# Autodesk Inventor assembly: power_pcb.brd
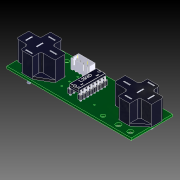
[picture p0: Inventor's stored thumbnail of the model, 180x180]
Saved by Autodesk Inventor 2020 (Build 240168000, 168)
## iProperties
Created: 2021-08-06
Part Number: power_pcb.brd
Document SubType Name: Assembly
Designer: Петров Иван
Mass: 15.8912 g
Surface Area: 154.202 cm^2
Volume: 15.8912 cm^3
Density: 1 g/cm^3
Author: Петров Иван
## Documents named in this file (6)
- E:\IVAN\Ivan_desktop\Kvantorium\Projects\RoboPatrol\electronic\COMMUATOR_POWER_PCB\power_pcb.brd.iam
- E:\IVAN\Ivan_desktop\Kvantorium\Projects\RoboPatrol\design\standart_components\BR05-PCB.ipt
- E:\IVAN\Ivan_desktop\Kvantorium\Projects\RoboPatrol\design\standart_components\SCSL-4.ipt
- E:\IVAN\Ivan_desktop\Kvantorium\Projects\RoboPatrol\design\standart_components\L293D v1.ipt
- E:\IVAN\Ivan_desktop\Kvantorium\Projects\RoboPatrol\design\standart_components\connectrs\JST - XH - Thru (V) - 4Pin - 2.54mm.ipt
- E:\IVAN\Ivan_desktop\Kvantorium\Projects\RoboPatrol\electronic\COMMUATOR_POWER_PCB\power_pcb.brdКонтур1.ipt
## Components (9 placed, 5 different names)
1. power_pcb.brdКонтур:2
2. BR05-PCB:1
3. BR05-PCB:2
4. L293D v1:1 — Совмещение:8, Совмещение:9
5. JST - XH - Thru (V) - 4Pin - 2.54mm:1
6. SCSL-4:1
7. SCSL-4:2 — Совмещение:8
8. SCSL-4:3
9. SCSL-4:4 — Совмещение:9
## Component patterns: (4 elements, first: SCSL-4:1)
## Relationships (15: Mate 12, Angle 3)
- [Mate]: power_pcb.brdКонтур:2 ↔ BR05-PCB:1
- [Mate]: power_pcb.brdКонтур:2 ↔ BR05-PCB:1
- [Angle] (-90 deg): power_pcb.brdКонтур:2 ↔ BR05-PCB:1
- [Mate]: power_pcb.brdКонтур:2 ↔ BR05-PCB:2
- [Mate]: power_pcb.brdКонтур:2 ↔ BR05-PCB:2
- [Angle] (0 deg): power_pcb.brdКонтур:2 ↔ BR05-PCB:2
- [Mate]: power_pcb.brdКонтур:2 ↔ SCSL-4:1
- [Mate]: power_pcb.brdКонтур:2 ↔ SCSL-4:1
- [Mate] (-0.3 mm): power_pcb.brdКонтур:2 ↔ SCSL-4:1
- Совмещение:8 [Mate] (0.5 mm): L293D v1:1 ↔ SCSL-4:2
- [Angle] (0 deg): power_pcb.brdКонтур:2 ↔ L293D v1:1
- Совмещение:9 [Mate]: L293D v1:1 ↔ SCSL-4:4
- [Mate]: power_pcb.brdКонтур:2 ↔ JST - XH - Thru (V) - 4Pin - 2.54mm:1
- [Mate]: power_pcb.brdКонтур:2 ↔ JST - XH - Thru (V) - 4Pin - 2.54mm:1
- [Mate]: power_pcb.brdКонтур:2 ↔ JST - XH - Thru (V) - 4Pin - 2.54mm:1
